# Autodesk Inventor assembly: zlozenieTymRazemOdwrotnie
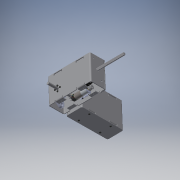
[picture p0: Inventor's stored thumbnail of the model, 180x180]
Saved by Autodesk Inventor 2019 (Build 230136000, 136)
## iProperties
Created: 2020-08-29
Part Number: zlozenieTymRazemOdwrotnie
Document SubType Name: Assembly
Designer: estee
Author: estee
## Documents named in this file (4)
- C:\Users\estee\OneDrive\Pulpit\estere\1\MUM\nowygit\Mechanika\Moduł obrotu DEK Bartek\odBartka\zlozenieTymRazemOdwrotnie.iam
- C:\Users\estee\OneDrive\Pulpit\estere\1\MUM\nowygit\Mechanika\Moduł obrotu DEK Bartek\odBartka\ObudowaNowa.iam
- C:\Users\estee\OneDrive\Pulpit\estere\1\MUM\nowygit\Mechanika\Moduł obrotu DEK Bartek\odBartka\ObudowaNowa2.iam
- C:\Users\estee\OneDrive\Dokumenty\Inventor\Content Center Files\R2019\en-US\ISO 4026\ISO 4026 - M3 x 3 - ISO.ipt
## Components (6 placed, 3 different names)
1. ObudowaNowa:1 [sub-assembly] — Mate:1, Angle:1, Mate:2, Tangent:1, Tangent:2, Tangent:3, Tangent:4
2. ObudowaNowa2:1 [sub-assembly] — Mate:1, Angle:1, Mate:2, Mate:3, Mate:4, Mate:5, Mate:6, Mate:7
3. ISO 4026 M3 x 3:1 — Mate:7, Tangent:4
4. ISO 4026 M3 x 3:2 — Mate:5, Tangent:3
5. ISO 4026 M3 x 3:3 — Mate:3, Mate:6, Tangent:1
6. ISO 4026 M3 x 3:4 — Mate:4, Tangent:2
## Relationships (12: Mate 7, Tangent 4, Angle 1)
- Mate:1: ObudowaNowa:1 ↔ ObudowaNowa2:1
- Angle:1 (0 deg): ObudowaNowa:1 ↔ ObudowaNowa2:1
- Mate:2 (5 mm): ObudowaNowa:1 ↔ ObudowaNowa2:1
- Mate:3: ObudowaNowa2:1 ↔ ISO 4026 M3 x 3:3
- Mate:4: ObudowaNowa2:1 ↔ ISO 4026 M3 x 3:4
- Mate:5: ObudowaNowa2:1 ↔ ISO 4026 M3 x 3:2
- Mate:6: ObudowaNowa2:1 ↔ ISO 4026 M3 x 3:3
- Tangent:1: ObudowaNowa:1 ↔ ISO 4026 M3 x 3:3
- Tangent:2: ObudowaNowa:1 ↔ ISO 4026 M3 x 3:4
- Tangent:3: ObudowaNowa:1 ↔ ISO 4026 M3 x 3:2
- Mate:7: ObudowaNowa2:1 ↔ ISO 4026 M3 x 3:1
- Tangent:4: ObudowaNowa:1 ↔ ISO 4026 M3 x 3:1
